# Autodesk Inventor assembly: DPLX_A003_Lab_Version_Small_RevB
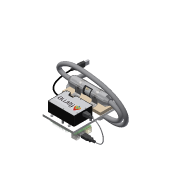
[picture p0: Inventor's stored thumbnail of the model, 180x180]
Saved by Autodesk Inventor 2018 (Build 220112000, 112)
## iProperties
Created: 2018-06-12
Part Number: DPLX_A003_Lab_Version_Small_RevB
Document SubType Name: Assembly
Designer: DPLXuser
Author: DPLXuser
## Documents named in this file (20)
- C:\Users\DPLXuser\Documents\GitHub\UMBC_DPLX_SPARK\SPARK CAD Files\DPLX_A003_Lab_Version_Small_RevB.iam
- C:\Users\DPLXuser\Documents\GitHub\UMBC_DPLX_SPARK\SPARK CAD Files\DPLX_P014_Lab_Baseplate_Small_PV.ipt
- C:\Users\DPLXuser\Documents\GitHub\UMBC_DPLX_SPARK\SPARK CAD Files\DPLX_P017_.5in _Standoff_smallplate.ipt
- C:\Users\DPLXuser\Documents\wire_t_to_b.ipt
- C:\Users\DPLXuser\Documents\GitHub\UMBC_DPLX_SPARK\SPARK CAD Files\DPLX_P021_Standoff_Rasp_pie_Lab_payload_sv.ipt
- C:\Users\DPLXuser\Documents\GitHub\UMBC_DPLX_SPARK\SPARK CAD Files\DPLX_A004_VIPE_Lab.iam
- C:\Users\DPLXuser\Documents\GitHub\UMBC_DPLX_SPARK\SPARK CAD Files\DPLX_P024_Ocean Optics Flame.iam
- C:\Users\DPLXuser\Documents\GitHub\UMBC_DPLX_SPARK\SPARK CAD Files\DPLX_A005_Spark_Gap_Lab.iam
- C:\Users\DPLXuser\Documents\GitHub\UMBC_DPLX_SPARK\SPARK CAD Files\DPLX_A006_RPi3.iam
- C:\Users\DPLXuser\Documents\GitHub\UMBC_DPLX_SPARK\SPARK CAD Files\91828A211_TYPE 18-8 STAINLESS STEEL HEX NUT.ipt
- C:\Users\DPLXuser\Documents\GitHub\UMBC_DPLX_SPARK\SPARK CAD Files\DPLX_P036 mini USB.ipt
- C:\Users\DPLXuser\Documents\GitHub\UMBC_DPLX_SPARK\SPARK CAD Files\DPLX_P037 USB.ipt
- C:\Users\DPLXuser\Documents\GitHub\UMBC_DPLX_SPARK\SPARK CAD Files\usb Wire.ipt
- C:\Users\DPLXuser\Documents\GitHub\UMBC_DPLX_SPARK\SPARK CAD Files\Wire to Spark Gap.ipt
- C:\Users\DPLXuser\Documents\GitHub\UMBC_DPLX_SPARK\SPARK CAD Files\Wire to Power.ipt
- C:\Users\DPLXuser\Documents\GitHub\UMBC_DPLX_SPARK\SPARK CAD Files\DPLX_P038 Micro USB.ipt
- C:\Users\DPLXuser\Documents\GitHub\UMBC_DPLX_SPARK\SPARK CAD Files\Pi Wire.ipt
- C:\Users\DPLXuser\Documents\GitHub\UMBC_DPLX_SPARK\SPARK CAD Files\Wire to Spark Gap 2.ipt
- C:\Users\DPLXuser\Documents\GitHub\UMBC_DPLX_SPARK\SPARK CAD Files\91772A115_18-8 SS PAN HEAD PHILLIPS MACHINE SCREW-01.ipt
- C:\Users\DPLXuser\Documents\GitHub\UMBC_DPLX_SPARK\SPARK CAD Files\91841A005_TYPE 18-8 STAINLESS STEEL HEX NUT.ipt
## Components (41 placed, 19 different names)
1. DPLX_P014_Lab_Baseplate_Small_PV:1 — Insert:1, Insert:2, Mate:23, Insert:36, Insert:37, Insert:51, Insert:52, Insert:55, Insert:56, Insert:58, Insert:60, Mate:24, Insert:63, Insert:64, Insert:65, Insert:66, Insert:67, Insert:68, Insert:69, Insert:70, Insert:85, Insert:86, Insert:87, Insert:94, Insert:95, Insert:96, Insert:97
2. DPLX_P017_.5in _Standoff_smallplate:2 — Insert:2, Insert:59
3. DPLX_P017_.5in _Standoff_smallplate:3 — Insert:1, Insert:57, Insert:58
4. DPLX_P017_.5in _Standoff_smallplate:4 — Mate:23
5. wire_t_to_b:1 — Flush:11, Flush:12
6. DPLX_P021_Standoff_Rasp_pie_Lab_payload_sv:2 — Insert:36
7. DPLX_P021_Standoff_Rasp_pie_Lab_payload_sv:3 — Insert:37
8. DPLX_P021_Standoff_Rasp_pie_Lab_payload_sv:6 — Insert:52
9. DPLX_P021_Standoff_Rasp_pie_Lab_payload_sv:7 — Insert:51
10. DPLX_A004_VIPE_Lab:1 [sub-assembly] — Insert:55, Insert:56, Insert:72, Mate:31, Flush:19
11. DPLX_P024_Ocean Optics Flame:1 [sub-assembly] — Insert:57, Insert:59, Insert:71
12. DPLX_A005_Spark_Gap_Lab:1 [sub-assembly] — Insert:60, Mate:24, Flush:16, Mate:32, Mate:33
13. DPLX_A006_RPi3:1 [sub-assembly] — Mate:25, Mate:27, Mate:28, Mate:30, Insert:90, Insert:91, Insert:92, Insert:93
14. 91828A211_TYPE 18-8 STAINLESS STEEL HEX NUT:1 — Insert:68
15. 91828A211_TYPE 18-8 STAINLESS STEEL HEX NUT:2 — Insert:70
16. 91828A211_TYPE 18-8 STAINLESS STEEL HEX NUT:3 — Insert:69
17. 91828A211_TYPE 18-8 STAINLESS STEEL HEX NUT:4 — Insert:66
18. 91828A211_TYPE 18-8 STAINLESS STEEL HEX NUT:5 — Insert:63
19. 91828A211_TYPE 18-8 STAINLESS STEEL HEX NUT:6 — Insert:67
20. 91828A211_TYPE 18-8 STAINLESS STEEL HEX NUT:7 — Insert:64
21. 91828A211_TYPE 18-8 STAINLESS STEEL HEX NUT:8 — Insert:65
22. DPLX_P036 mini USB:1 — Insert:71, Flush:13, Mate:26
23. DPLX_P037 USB:1 — Mate:25, Flush:14
24. usb Wire:1 — Flush:13, Flush:14, Mate:26
25. Wire to Spark Gap:1 — Flush:15, Flush:16
26. Wire to Power:1 — Insert:72, Mate:29
27. DPLX_P038 Micro USB:1 — Mate:27, Mate:28, Flush:17
28. Pi Wire:1 — Flush:17, Mate:29, Mate:30, Insert:73
29. DPLX_P037 USB:2 — Insert:73
30. Wire to Spark Gap 2:1 — Flush:18, Flush:19
31. 91772A115_18-8 SS PAN HEAD PHILLIPS MACHINE SCREW-01:1 — Insert:85
32. 91772A115_18-8 SS PAN HEAD PHILLIPS MACHINE SCREW-01:2 — Insert:86
33. 91772A115_18-8 SS PAN HEAD PHILLIPS MACHINE SCREW-01:3 — Insert:87
34. 91772A115_18-8 SS PAN HEAD PHILLIPS MACHINE SCREW-01:4 — Insert:91
35. 91772A115_18-8 SS PAN HEAD PHILLIPS MACHINE SCREW-01:5 — Insert:93
36. 91772A115_18-8 SS PAN HEAD PHILLIPS MACHINE SCREW-01:6 — Insert:90
37. 91772A115_18-8 SS PAN HEAD PHILLIPS MACHINE SCREW-01:7 — Insert:92
38. 91841A005_TYPE 18-8 STAINLESS STEEL HEX NUT:1 — Insert:95
39. 91841A005_TYPE 18-8 STAINLESS STEEL HEX NUT:2 — Insert:94
40. 91841A005_TYPE 18-8 STAINLESS STEEL HEX NUT:3 — Insert:96
41. 91841A005_TYPE 18-8 STAINLESS STEEL HEX NUT:4 — Insert:97
## Relationships (54: Insert 34, Mate 11, Flush 9)
- Insert:1: DPLX_P014_Lab_Baseplate_Small_PV:1 ↔ DPLX_P017_.5in _Standoff_smallplate:3
- Insert:2: DPLX_P014_Lab_Baseplate_Small_PV:1 ↔ DPLX_P017_.5in _Standoff_smallplate:2
- Mate:23: DPLX_P014_Lab_Baseplate_Small_PV:1 ↔ DPLX_P017_.5in _Standoff_smallplate:4
- Flush:11: wire_t_to_b:1
- Flush:12: wire_t_to_b:1
- Insert:36: DPLX_P014_Lab_Baseplate_Small_PV:1 ↔ DPLX_P021_Standoff_Rasp_pie_Lab_payload_sv:2
- Insert:37: DPLX_P014_Lab_Baseplate_Small_PV:1 ↔ DPLX_P021_Standoff_Rasp_pie_Lab_payload_sv:3
- Insert:51: DPLX_P014_Lab_Baseplate_Small_PV:1 ↔ DPLX_P021_Standoff_Rasp_pie_Lab_payload_sv:7
- Insert:52: DPLX_P014_Lab_Baseplate_Small_PV:1 ↔ DPLX_P021_Standoff_Rasp_pie_Lab_payload_sv:6
- Insert:55: DPLX_P014_Lab_Baseplate_Small_PV:1 ↔ DPLX_A004_VIPE_Lab:1
- Insert:56: DPLX_P014_Lab_Baseplate_Small_PV:1 ↔ DPLX_A004_VIPE_Lab:1
- Insert:57: DPLX_P017_.5in _Standoff_smallplate:3 ↔ DPLX_P024_Ocean Optics Flame:1
- Insert:58: DPLX_P014_Lab_Baseplate_Small_PV:1 ↔ DPLX_P017_.5in _Standoff_smallplate:3
- Insert:59: DPLX_P017_.5in _Standoff_smallplate:2 ↔ DPLX_P024_Ocean Optics Flame:1
- Insert:60: DPLX_P014_Lab_Baseplate_Small_PV:1 ↔ DPLX_A005_Spark_Gap_Lab:1
- Mate:24: DPLX_P014_Lab_Baseplate_Small_PV:1 ↔ DPLX_A005_Spark_Gap_Lab:1
- Insert:63: DPLX_P014_Lab_Baseplate_Small_PV:1 ↔ 91828A211_TYPE 18-8 STAINLESS STEEL HEX NUT:5
- Insert:64: DPLX_P014_Lab_Baseplate_Small_PV:1 ↔ 91828A211_TYPE 18-8 STAINLESS STEEL HEX NUT:7
- Insert:65: DPLX_P014_Lab_Baseplate_Small_PV:1 ↔ 91828A211_TYPE 18-8 STAINLESS STEEL HEX NUT:8
- Insert:66: DPLX_P014_Lab_Baseplate_Small_PV:1 ↔ 91828A211_TYPE 18-8 STAINLESS STEEL HEX NUT:4
- Insert:67: DPLX_P014_Lab_Baseplate_Small_PV:1 ↔ 91828A211_TYPE 18-8 STAINLESS STEEL HEX NUT:6
- Insert:68: DPLX_P014_Lab_Baseplate_Small_PV:1 ↔ 91828A211_TYPE 18-8 STAINLESS STEEL HEX NUT:1
- Insert:69: DPLX_P014_Lab_Baseplate_Small_PV:1 ↔ 91828A211_TYPE 18-8 STAINLESS STEEL HEX NUT:3
- Insert:70: DPLX_P014_Lab_Baseplate_Small_PV:1 ↔ 91828A211_TYPE 18-8 STAINLESS STEEL HEX NUT:2
- Insert:71 (-7.62 mm): DPLX_P024_Ocean Optics Flame:1 ↔ DPLX_P036 mini USB:1
- Mate:25: DPLX_A006_RPi3:1 ↔ DPLX_P037 USB:1
- Flush:13: DPLX_P036 mini USB:1 ↔ usb Wire:1
- Flush:14: DPLX_P037 USB:1 ↔ usb Wire:1
- Mate:26: DPLX_P036 mini USB:1 ↔ usb Wire:1
- Flush:15: Wire to Spark Gap:1
- Flush:16: DPLX_A005_Spark_Gap_Lab:1 ↔ Wire to Spark Gap:1
- Insert:72: DPLX_A004_VIPE_Lab:1 ↔ Wire to Power:1
- Mate:27: DPLX_A006_RPi3:1 ↔ DPLX_P038 Micro USB:1
- Mate:28: DPLX_A006_RPi3:1 ↔ DPLX_P038 Micro USB:1
- Flush:17: DPLX_P038 Micro USB:1 ↔ Pi Wire:1
- Mate:29: Wire to Power:1 ↔ Pi Wire:1
- Mate:30: DPLX_A006_RPi3:1 ↔ Pi Wire:1
- Insert:73: Pi Wire:1 ↔ DPLX_P037 USB:2
- Mate:31: DPLX_A004_VIPE_Lab:1
- Mate:32: DPLX_A005_Spark_Gap_Lab:1
- Mate:33: DPLX_A005_Spark_Gap_Lab:1
- Flush:18: Wire to Spark Gap 2:1
- Flush:19: DPLX_A004_VIPE_Lab:1 ↔ Wire to Spark Gap 2:1
- Insert:85: DPLX_P014_Lab_Baseplate_Small_PV:1 ↔ 91772A115_18-8 SS PAN HEAD PHILLIPS MACHINE SCREW-01:1
- Insert:86: DPLX_P014_Lab_Baseplate_Small_PV:1 ↔ 91772A115_18-8 SS PAN HEAD PHILLIPS MACHINE SCREW-01:2
- Insert:87: DPLX_P014_Lab_Baseplate_Small_PV:1 ↔ 91772A115_18-8 SS PAN HEAD PHILLIPS MACHINE SCREW-01:3
- Insert:90: DPLX_A006_RPi3:1 ↔ 91772A115_18-8 SS PAN HEAD PHILLIPS MACHINE SCREW-01:6
- Insert:91: DPLX_A006_RPi3:1 ↔ 91772A115_18-8 SS PAN HEAD PHILLIPS MACHINE SCREW-01:4
- Insert:92: DPLX_A006_RPi3:1 ↔ 91772A115_18-8 SS PAN HEAD PHILLIPS MACHINE SCREW-01:7
- Insert:93: DPLX_A006_RPi3:1 ↔ 91772A115_18-8 SS PAN HEAD PHILLIPS MACHINE SCREW-01:5
- Insert:94: DPLX_P014_Lab_Baseplate_Small_PV:1 ↔ 91841A005_TYPE 18-8 STAINLESS STEEL HEX NUT:2
- Insert:95: DPLX_P014_Lab_Baseplate_Small_PV:1 ↔ 91841A005_TYPE 18-8 STAINLESS STEEL HEX NUT:1
- Insert:96: DPLX_P014_Lab_Baseplate_Small_PV:1 ↔ 91841A005_TYPE 18-8 STAINLESS STEEL HEX NUT:3
- Insert:97: DPLX_P014_Lab_Baseplate_Small_PV:1 ↔ 91841A005_TYPE 18-8 STAINLESS STEEL HEX NUT:4
